# Autodesk Inventor assembly: CanSat Assembly
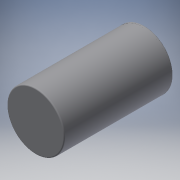
[picture p0: Inventor's stored thumbnail of the model, 180x180]
Saved by Autodesk Inventor 2018 (Build 220112000, 112)
## iProperties
Created: 2018-03-22
Part Number: CanSat Assembly
Document SubType Name: Assembly
Designer: boeingnut
Author: boeingnut
## Documents named in this file (3)
- C:\Users\boeingnut\Documents\CanSat\CanSat Assembly.iam
- C:\Users\boeingnut\Documents\CanSat\CanSatHousing.ipt
- C:\Users\boeingnut\Documents\CanSat\CanSat Cap.ipt
## Components (2 placed, 2 different names)
1. CanSatHousing:1 — Flush:1
2. CanSat Cap:1 — Flush:1
## Relationships (1: Flush 1)
- Flush:1: CanSatHousing:1 ↔ CanSat Cap:1
